# Autodesk Inventor assembly: kraken-power-adapter 1
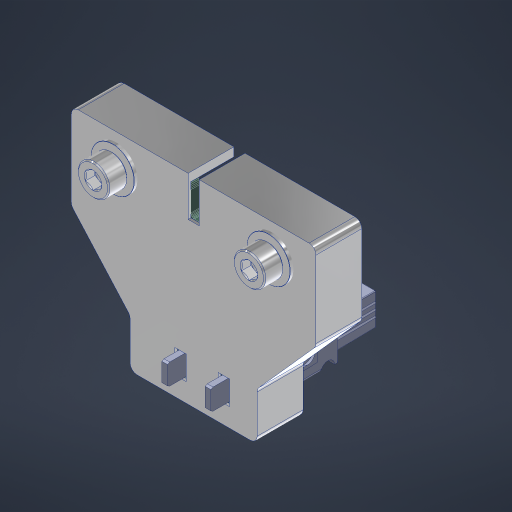
[picture p0: Inventor's stored thumbnail of the model, 512x512]
Saved by Autodesk Inventor 2023.3 (Build 273359000, 359)
## iProperties
Company: Kicad
Created: 2023-12-28
Part Number: kraken-power-adapter 1
Description: KiCad electronic assembly
Document SubType Name: Assembly
Designer: mavericks
Authority: Unknown
Sending System: KiCad to STEP converter
Preprocessor: Open CASCADE STEP processor 7.5
Title: kraken-power-adapter.step
Author: Pcbnew
## Documents named in this file (6)
- C:\Users\mavericks\Desktop\Crescendo_2024-CAD\2024 Robot\COMMON PARTS\MOTORS\Kracken\kraken-power-adapter.iam
- C:\Users\mavericks\Desktop\Crescendo_2024-CAD\2024 Robot\COMMON PARTS\MOTORS\Kracken\92916A325_Brass Washer.iam
- C:\Users\mavericks\Desktop\Crescendo_2024-CAD\2024 Robot\COMMON PARTS\MOTORS\Kracken\93465A147_Brass Socket Head Screw.iam
- C:\Users\mavericks\Desktop\Crescendo_2024-CAD\2024 Robot\COMMON PARTS\MOTORS\Kracken\1335G1 IN HSG.iam
- C:\Users\mavericks\Desktop\Crescendo_2024-CAD\2024 Robot\COMMON PARTS\MOTORS\Kracken\kraken-power-adapter PCB.ipt
- C:\Users\mavericks\Desktop\Crescendo_2024-CAD\2024 Robot\COMMON PARTS\MOTORS\Kracken\kracken Cover.ipt
## Components (8 placed, 8 different names)
1. 2 [sub-assembly]
2. 4 [sub-assembly]
3. 5 [sub-assembly]
4. 6 [sub-assembly]
5. 8 [sub-assembly]
6. 9 [sub-assembly]
7. 10 — Mate:1, Mate:2, Mate:3
8. kracken Cover:1 — Mate:1, Mate:2, Mate:3
## Relationships (3: Mate 3)
- Mate:1: 10 ↔ kracken Cover:1
- Mate:2: 10 ↔ kracken Cover:1
- Mate:3: 10 ↔ kracken Cover:1
